# Autodesk Inventor assembly: bottom box with container
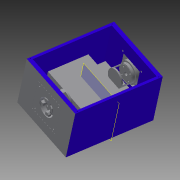
[picture p0: Inventor's stored thumbnail of the model, 180x180]
Saved by Autodesk Inventor 2015 (Build 190159000, 159)
## iProperties
Created: 2014-09-09
Part Number: bottom box with container
Document SubType Name: Assembly
Designer: ericd_000
Author: ericd_000
## Documents named in this file (9)
- C:\Users\ericd_000\Dropbox\GitHub\initial_cad\eric_cad\bottom box with container.iam
- C:\Users\ericd_000\Dropbox\GitHub\initial_cad\eric_cad\bayonet container.ipt
- C:\Users\ericd_000\Dropbox\GitHub\initial_cad\eric_cad\brain box bottom.ipt
- C:\Users\ericd_000\Dropbox\GitHub\initial_cad\eric_cad\bbb brick.ipt
- C:\Users\ericd_000\Dropbox\GitHub\initial_cad\eric_cad\battery pack.ipt
- C:\Users\ericd_000\Dropbox\GitHub\initial_cad\eric_cad\usb hub d link.ipt
- C:\Users\ericd_000\Dropbox\GitHub\initial_cad\eric_cad\ankerpro15000mah.ipt
- C:\Users\ericd_000\Dropbox\GitHub\initial_cad\eric_cad\intocircuit 26Ah.ipt
- C:\Users\ericd_000\Dropbox\GitHub\initial_cad\eric_cad\udoo.ipt
## Components (10 placed, 8 different names)
1. brain box bottom:1 — Rigid:1, Rotational:1, Rotational:2, Mate:1, Mate:2, Mate:3, Mate:4, Mate:5, Mate:6, Mate:7, Mate:9, Mate:11, Mate:12, Mate:13, Mate:14
2. bayonet container:2 — Rigid:1
3. bayonet container:3 — Rotational:1, Mate:4
4. bbb brick:1 — Mate:1, Mate:2
5. bayonet container:4 — Rotational:2, Mate:3, Mate:8, Mate:10
6. battery pack:1 — Mate:5
7. usb hub d link:1 — Mate:6, Mate:7
8. ankerpro15000mah:1 — Mate:8, Mate:9
9. intocircuit 26Ah:1 — Mate:10, Mate:11
10. udoo:1 — Mate:12, Mate:13, Mate:14
## Relationships (17: Mate 14, RevoluteJoint 2, WeldJoint 1)
- Rigid:1 [WeldJoint]: brain box bottom:1 ↔ bayonet container:2
- Rotational:1 [RevoluteJoint]: brain box bottom:1 ↔ bayonet container:3
- Rotational:2 [RevoluteJoint]: brain box bottom:1 ↔ bayonet container:4
- Mate:1: brain box bottom:1 ↔ bbb brick:1
- Mate:2 (2.54 mm): brain box bottom:1 ↔ bbb brick:1
- Mate:3: brain box bottom:1 ↔ bayonet container:4
- Mate:4: brain box bottom:1 ↔ bayonet container:3
- Mate:5: brain box bottom:1 ↔ battery pack:1
- Mate:6: brain box bottom:1 ↔ usb hub d link:1
- Mate:7 (2.54 mm): brain box bottom:1 ↔ usb hub d link:1
- Mate:8 (2.54 mm): bayonet container:4 ↔ ankerpro15000mah:1
- Mate:9 (2.54 mm): brain box bottom:1 ↔ ankerpro15000mah:1
- Mate:10 (7.62 mm): bayonet container:4 ↔ intocircuit 26Ah:1
- Mate:11 (5.08 mm): brain box bottom:1 ↔ intocircuit 26Ah:1
- Mate:12: brain box bottom:1 ↔ udoo:1
- Mate:13 (1.27 mm): brain box bottom:1 ↔ udoo:1
- Mate:14 (2.54 mm): brain box bottom:1 ↔ udoo:1
